# Autodesk Inventor assembly: steam cylinder 1
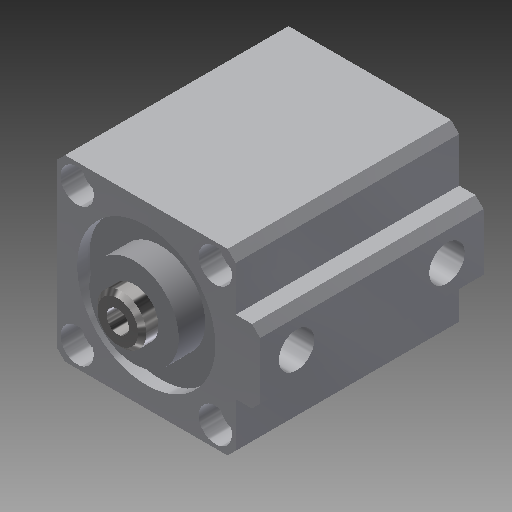
[picture p0: Inventor's stored thumbnail of the model, 512x512]
Saved by Autodesk Inventor 2017 SP1 (Build 210196100, 196)
## iProperties
Created: 2017-06-14
Part Number: steam cylinder 1
Document SubType Name: Assembly
Designer: RMcComber
Author: RMcComber
## Documents named in this file (4)
- C:\Users\rmccomber\Documents\st motor\two cylinder spool valve\steam cylinder 1.iam
- C:\Users\rmccomber\Documents\st motor\two cylinder spool valve\cylinder.ipt
- C:\Users\rmccomber\Documents\st motor\two cylinder spool valve\piston.ipt
- C:\Users\rmccomber\Documents\st motor\two cylinder spool valve\cylinder cap.ipt
## Components (3 placed, 3 different names)
1. cylinder:1 — Mate:1, Flush:1, Mate:2, Flush:2
2. piston:1 — Mate:1, Flush:1
3. cylinder cap:1 — Mate:2, Flush:2
## Relationships (4: Mate 2, Flush 2)
- Mate:1: cylinder:1 ↔ piston:1
- Flush:1 (-7 mm): cylinder:1 ↔ piston:1
- Mate:2: cylinder:1 ↔ cylinder cap:1
- Flush:2 (-3 mm): cylinder:1 ↔ cylinder cap:1
